# Autodesk Inventor assembly: kinematic-mount-assembly
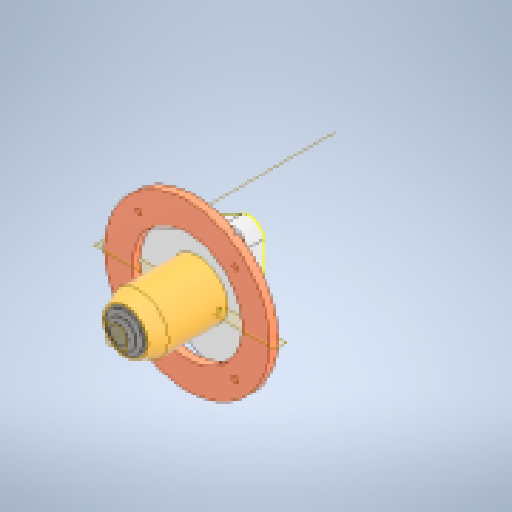
[picture p0: Inventor's stored thumbnail of the model, 512x512]
Saved by Autodesk Inventor 2026.1 (Build 301233000, 233)
## iProperties
Created: 2019-02-14
Part Number: kinematic-mount-assembly
Document SubType Name: Assembly
Designer: rainer
Author: rainer
## Documents named in this file (6)
- C:\Users\user\Desktop\setup for publishing\kinematic-mount-assembly.iam
- C:\Users\user\Desktop\setup for publishing\kinematic-mount_base.ipt
- C:\Users\user\Desktop\setup for publishing\Triangle_RK.ipt
- C:\Users\user\Desktop\setup for publishing\F6MSS12-Step.ipt
- C:\Users\user\Desktop\setup for publishing\Nikon-Objektive-MUC11900_Mockup.ipt
- C:\Users\user\Desktop\setup for publishing\Nikon-Objective-Insulation_singe_cable_grooves_v2.ipt
## Components (7 placed, 5 different names)
1. kinematic-mount_base:1 — Passend:1, Passend:5, Passend:6
2. Triangle_RK:1 — Passend:1, Passend:2, Fluchtend:1, Passend:3, Fluchtend:2, Passend:4, Fluchtend:3, Passend:6, Passend:9, Passend:12
3. F6MSS12-Step:1 — Passend:4, Fluchtend:3
4. F6MSS12-Step:2 — Passend:3, Fluchtend:2
5. F6MSS12-Step:3 — Passend:2, Fluchtend:1, Passend:5
6. Nikon-Objektive-MUC11900_Mockup:1 — Passend:9, Fluchtend:4, Passend:12
7. Nikon-Objective-Insulation_singe_cable_grooves_v2:1 — Fluchtend:4
## Relationships (12: Mate 8, Flush 4)
- Passend:1 [Mate]: kinematic-mount_base:1 ↔ Triangle_RK:1
- Passend:2 [Mate]: Triangle_RK:1 ↔ F6MSS12-Step:3
- Fluchtend:1 [Flush] (4 mm): Triangle_RK:1 ↔ F6MSS12-Step:3
- Passend:3 [Mate]: Triangle_RK:1 ↔ F6MSS12-Step:2
- Fluchtend:2 [Flush] (4 mm): Triangle_RK:1 ↔ F6MSS12-Step:2
- Passend:4 [Mate]: Triangle_RK:1 ↔ F6MSS12-Step:1
- Fluchtend:3 [Flush] (4 mm): Triangle_RK:1 ↔ F6MSS12-Step:1
- Passend:5 [Mate] (0.5 mm): kinematic-mount_base:1 ↔ F6MSS12-Step:3
- Passend:6 [Mate]: kinematic-mount_base:1 ↔ Triangle_RK:1
- Passend:9 [Mate]: Triangle_RK:1 ↔ Nikon-Objektive-MUC11900_Mockup:1
- Fluchtend:4 [Flush]: Nikon-Objektive-MUC11900_Mockup:1 ↔ Nikon-Objective-Insulation_singe_cable_grooves_v2:1
- Passend:12 [Mate]: Triangle_RK:1 ↔ Nikon-Objektive-MUC11900_Mockup:1
